# Autodesk Inventor assembly: TR2 Arm
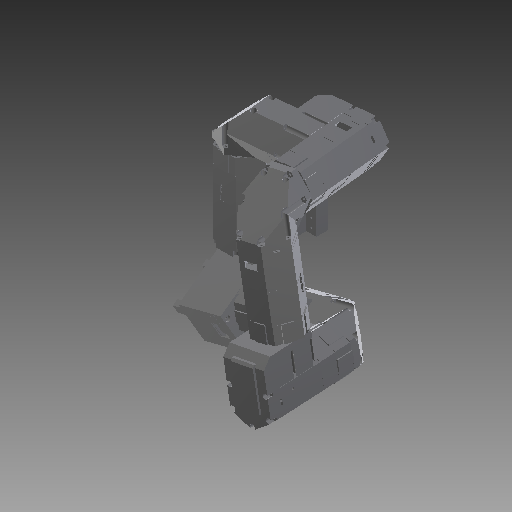
[picture p0: Inventor's stored thumbnail of the model, 512x512]
Saved by Autodesk Inventor 2017 (Build 210142000, 142)
## iProperties
Created: 2018-10-11
Part Number: TR2 Arm
Document SubType Name: Assembly
Designer: Zach
Author: Zach
## Documents named in this file (7)
- C:\Users\Dell\Documents\GitHub\tr2\Arm\Arm.iam
- C:\Users\Dell\Documents\GitHub\tr2\Gripper\Gripper.iam
- C:\Users\Dell\Documents\GitHub\tr2\Arm\TARM09b.ipt
- C:\Users\Dell\Documents\GitHub\tr2\Arm\TARM01b.ipt
- C:\Users\Dell\Documents\GitHub\tr2\Arm\TARM02b.ipt
- C:\Users\Dell\Documents\GitHub\tr2\Arm\TARM14.ipt
- C:\Users\Dell\Documents\GitHub\tr2\Actuator 1.3\Actuator 1.3.iam
## Components (12 placed, 6 different names)
1. TARM01b:1 — Mate:241, Mate:242, Mate:243, Mate:244, Mate:245, Mate:246, Mate:269
2. Gripper:1 [sub-assembly] — Mate:267, Mate:268
3. TARM09b:1 — Mate:186, Mate:187, Mate:188, Mate:249, Mate:250, Mate:251
4. TARM09b:2 — Mate:257, Mate:258, Mate:259, Mate:260, Mate:261
5. TARM02b:1 — Mate:186, Mate:187, Mate:188, Mate:247, Mate:248
6. TARM14:1 — Mate:252, Mate:253, Mate:254, Mate:255, Mate:256
7. TARM14:2 — Mate:262, Mate:263, Mate:264, Mate:265, Mate:266
8. Actuator 1.3:1 [sub-assembly] — Mate:244, Mate:245, Mate:246, Mate:247, Mate:248, Mate:269
9. Actuator 1.3:2 [sub-assembly] — Mate:249, Mate:250, Mate:251, Mate:252, Mate:253
10. Actuator 1.3:3 [sub-assembly] — Mate:254, Mate:255, Mate:256, Mate:257, Mate:258
11. Actuator 1.3:4 [sub-assembly] — Mate:259, Mate:260, Mate:261, Mate:262, Mate:263
12. Actuator 1.3:5 [sub-assembly] — Mate:264, Mate:265, Mate:266, Mate:267, Mate:268
## Relationships (32: Mate 32)
- Mate:186: TARM09b:1 ↔ TARM02b:1
- Mate:187: TARM09b:1 ↔ TARM02b:1
- Mate:188: TARM09b:1 ↔ TARM02b:1
- Mate:241: TARM01b:1
- Mate:242: TARM01b:1
- Mate:243: TARM01b:1
- Mate:244: TARM01b:1 ↔ Actuator 1.3:1
- Mate:245: TARM01b:1 ↔ Actuator 1.3:1
- Mate:246: TARM01b:1 ↔ Actuator 1.3:1
- Mate:247: TARM02b:1 ↔ Actuator 1.3:1
- Mate:248: TARM02b:1 ↔ Actuator 1.3:1
- Mate:249: TARM09b:1 ↔ Actuator 1.3:2
- Mate:250: TARM09b:1 ↔ Actuator 1.3:2
- Mate:251: TARM09b:1 ↔ Actuator 1.3:2
- Mate:252: TARM14:1 ↔ Actuator 1.3:2
- Mate:253: TARM14:1 ↔ Actuator 1.3:2
- Mate:254: TARM14:1 ↔ Actuator 1.3:3
- Mate:255: TARM14:1 ↔ Actuator 1.3:3
- Mate:256: TARM14:1 ↔ Actuator 1.3:3
- Mate:257: TARM09b:2 ↔ Actuator 1.3:3
- Mate:258: TARM09b:2 ↔ Actuator 1.3:3
- Mate:259: TARM09b:2 ↔ Actuator 1.3:4
- Mate:260: TARM09b:2 ↔ Actuator 1.3:4
- Mate:261: TARM09b:2 ↔ Actuator 1.3:4
- Mate:262: TARM14:2 ↔ Actuator 1.3:4
- Mate:263: TARM14:2 ↔ Actuator 1.3:4
- Mate:264: TARM14:2 ↔ Actuator 1.3:5
- Mate:265: TARM14:2 ↔ Actuator 1.3:5
- Mate:266: TARM14:2 ↔ Actuator 1.3:5
- Mate:267: Gripper:1 ↔ Actuator 1.3:5
- Mate:268: Gripper:1 ↔ Actuator 1.3:5
- Mate:269: TARM01b:1 ↔ Actuator 1.3:1
